# Autodesk Inventor assembly: Full_Assembly
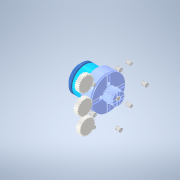
[picture p0: Inventor's stored thumbnail of the model, 180x180]
Saved by Autodesk Inventor 2022 (Build 260153000, 153)
## iProperties
Created: 2022-04-22
Part Number: Full_Assembly
Document SubType Name: Assembly
Designer: Mlees
Author: Mlees
## Documents named in this file (7)
- C:\Users\Mlees\Desktop\504Engineering\Project_0000\Designs\Design_2\Created_Parts\Full_Assembly.iam
- C:\Users\Mlees\Desktop\504Engineering\Project_0000\Designs\Design_2\Created_Parts\Gear_Box_Chasis_Lvl_1.ipt
- C:\Users\Mlees\Desktop\504Engineering\Project_0000\Designs\Design_2\Downloads\94180A323_Tapered Heat-Set Inserts_M2-5x0-45x5-6_9-64inmaxholesize.ipt
- C:\Users\Mlees\Desktop\504Engineering\Project_0000\Designs\Design_2\Created_Parts\Gear_Box_Chasis_Divider.ipt
- C:\Users\Mlees\Desktop\504Engineering\Project_0000\Designs\Design_2\Created_Parts\Gear_Box_Motor_Input.ipt
- C:\Users\Mlees\Desktop\504Engineering\Project_0000\Designs\Design_2\Downloads\m100-motor-1.snapshot.1\M100-MOTOR-R1.ipt
- C:\Users\Mlees\Desktop\504Engineering\Project_0000\Designs\Design_2\Created_Parts\Gear_Folder\5to1GearCreation_Trial_1\Design Accelerator\Spur Gear23.ipt
## Components (15 placed, 5 different names)
1. Spur Gear2:1 — Mate:1, Mate:2, Mate:3, Mate:4, Mate:5, Mate:6, Mate:7, Mate:8, Mate:9, Mate:10, Mate:11, Mate:12, Mate:13, Mate:14, Mate:15, Mate:16, Mate:17, Mate:18, Mate:24, Mate:25
2. 94180A323_Tapered Heat-Set Inserts_M2-5x0-45x5-6_9-64inmaxholesize:1 — Mate:9, Mate:10
3. 94180A323_Tapered Heat-Set Inserts_M2-5x0-45x5-6_9-64inmaxholesize:2 — Mate:13, Mate:14
4. 94180A323_Tapered Heat-Set Inserts_M2-5x0-45x5-6_9-64inmaxholesize:3 — Mate:5, Mate:6
5. 94180A323_Tapered Heat-Set Inserts_M2-5x0-45x5-6_9-64inmaxholesize:4 — Mate:7, Mate:8, Mate:19
6. 94180A323_Tapered Heat-Set Inserts_M2-5x0-45x5-6_9-64inmaxholesize:5 — Mate:3, Mate:4
7. 94180A323_Tapered Heat-Set Inserts_M2-5x0-45x5-6_9-64inmaxholesize:6 — Mate:1, Mate:2
8. 94180A323_Tapered Heat-Set Inserts_M2-5x0-45x5-6_9-64inmaxholesize:7 — Mate:11, Mate:12
9. 94180A323_Tapered Heat-Set Inserts_M2-5x0-45x5-6_9-64inmaxholesize:8 — Mate:15, Mate:16
10. Gear_Box_Chasis_Divider:1 — Mate:17, Mate:18, Mate:19
11. Spur Gear1:1 — Mate:20, Mate:23, Mate:21, Mate:24, Mate:25
12. M100-MOTOR-R1:1 — Mate:20, Mate:23, Mate:21
13. Spur Gear2:2
14. Spur Gear2:3
15. Spur Gear2:4
## Relationships (24: Mate 24)
- Mate:1: Spur Gear2:1 ↔ 94180A323_Tapered Heat-Set Inserts_M2-5x0-45x5-6_9-64inmaxholesize:6
- Mate:2: Spur Gear2:1 ↔ 94180A323_Tapered Heat-Set Inserts_M2-5x0-45x5-6_9-64inmaxholesize:6
- Mate:3: Spur Gear2:1 ↔ 94180A323_Tapered Heat-Set Inserts_M2-5x0-45x5-6_9-64inmaxholesize:5
- Mate:4: Spur Gear2:1 ↔ 94180A323_Tapered Heat-Set Inserts_M2-5x0-45x5-6_9-64inmaxholesize:5
- Mate:5: Spur Gear2:1 ↔ 94180A323_Tapered Heat-Set Inserts_M2-5x0-45x5-6_9-64inmaxholesize:3
- Mate:6: Spur Gear2:1 ↔ 94180A323_Tapered Heat-Set Inserts_M2-5x0-45x5-6_9-64inmaxholesize:3
- Mate:7: Spur Gear2:1 ↔ 94180A323_Tapered Heat-Set Inserts_M2-5x0-45x5-6_9-64inmaxholesize:4
- Mate:8: Spur Gear2:1 ↔ 94180A323_Tapered Heat-Set Inserts_M2-5x0-45x5-6_9-64inmaxholesize:4
- Mate:9: Spur Gear2:1 ↔ 94180A323_Tapered Heat-Set Inserts_M2-5x0-45x5-6_9-64inmaxholesize:1
- Mate:10: Spur Gear2:1 ↔ 94180A323_Tapered Heat-Set Inserts_M2-5x0-45x5-6_9-64inmaxholesize:1
- Mate:11: Spur Gear2:1 ↔ 94180A323_Tapered Heat-Set Inserts_M2-5x0-45x5-6_9-64inmaxholesize:7
- Mate:12: Spur Gear2:1 ↔ 94180A323_Tapered Heat-Set Inserts_M2-5x0-45x5-6_9-64inmaxholesize:7
- Mate:13: Spur Gear2:1 ↔ 94180A323_Tapered Heat-Set Inserts_M2-5x0-45x5-6_9-64inmaxholesize:2
- Mate:14: Spur Gear2:1 ↔ 94180A323_Tapered Heat-Set Inserts_M2-5x0-45x5-6_9-64inmaxholesize:2
- Mate:15: Spur Gear2:1 ↔ 94180A323_Tapered Heat-Set Inserts_M2-5x0-45x5-6_9-64inmaxholesize:8
- Mate:16: Spur Gear2:1 ↔ 94180A323_Tapered Heat-Set Inserts_M2-5x0-45x5-6_9-64inmaxholesize:8
- Mate:17: Spur Gear2:1 ↔ Gear_Box_Chasis_Divider:1
- Mate:18: Spur Gear2:1 ↔ Gear_Box_Chasis_Divider:1
- Mate:19: 94180A323_Tapered Heat-Set Inserts_M2-5x0-45x5-6_9-64inmaxholesize:4 ↔ Gear_Box_Chasis_Divider:1
- Mate:20: Spur Gear1:1 ↔ M100-MOTOR-R1:1
- Mate:23: Spur Gear1:1 ↔ M100-MOTOR-R1:1
- Mate:21: Spur Gear1:1 ↔ M100-MOTOR-R1:1
- Mate:24: Spur Gear2:1 ↔ Spur Gear1:1
- Mate:25: Spur Gear2:1 ↔ Spur Gear1:1
